# Autodesk Inventor assembly: Tamale - V1
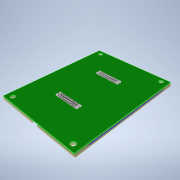
[picture p0: Inventor's stored thumbnail of the model, 180x180]
Saved by Autodesk Inventor 2022 (Build 260153000, 153)
## iProperties
Created: 2022-02-01
Part Number: Tamale - V1
Document SubType Name: Assembly
Designer: Caleb
Author: Caleb
## Documents named in this file (6)
- C:\Users\Caleb\Desktop\nebraska-silicon-lab\Hardware\ETL\modules\tamale\Tamale - V1p1.iam
- C:\Users\Caleb\Desktop\nebraska-silicon-lab\Hardware\ETL\modules\etl standard baseplate with cutouts.ipt
- C:\Users\Caleb\Desktop\nebraska-silicon-lab\Hardware\ETL\modules\tamale\BBM.iam
- C:\Users\Caleb\Desktop\nebraska-silicon-lab\Hardware\ETL\modules\tamale\Wirebond.ipt
- C:\Users\Caleb\Desktop\nebraska-silicon-lab\Hardware\ETL\modules\tamale\Mock Module PCB - V2p1.iam
- C:\Users\Caleb\Desktop\nebraska-silicon-lab\Hardware\ETL\modules\tamale\Short Wirebond.ipt
## Components (290 placed, 5 different names)
1. etl standard baseplate with cutouts:1 — Mate:7, Flush:5, Flush:6
2. BBM:1 [sub-assembly] — Mate:2, Angle:2, Flush:1, Flush:4, Mate:5, Mate:7, Mate:8
3. BBM:2 [sub-assembly] — Mate:3, Angle:1, Flush:2, Flush:4
4. BBM:3 [sub-assembly] — Mate:1, Angle:3, Flush:1, Flush:3, Mate:5, Mate:6
5. BBM:4 [sub-assembly] — Mate:4, Angle:4, Flush:2, Flush:3, Mate:6
6. Mock Module PCB - V2p1:1 [sub-assembly] — Mate:1, Mate:2, Mate:3, Mate:4, Angle:1, Angle:2, Angle:3, Angle:4, Flush:5, Flush:6
7. Wirebond:1 — Mate:8
8. Wirebond:2
9. Wirebond:3
10. Wirebond:4
11. Wirebond:5
12. Wirebond:6
13. Wirebond:7
14. Wirebond:8
15. Wirebond:9
16. Wirebond:10
17. Wirebond:11
18. Wirebond:12
19. Wirebond:13
20. Wirebond:14
21. Wirebond:15
22. Wirebond:16
23. Wirebond:17
24. Wirebond:18
25. Wirebond:19
26. Wirebond:20
27. Wirebond:21
28. Wirebond:22
29. Wirebond:23
30. Wirebond:24
31. Wirebond:25
32. Wirebond:26
33. Wirebond:27
34. Wirebond:28
35. Wirebond:29
36. Wirebond:30
37. Wirebond:31
38. Wirebond:32
39. Wirebond:33
40. Wirebond:34
41. Wirebond:35
42. Wirebond:36
43. Wirebond:37
44. Wirebond:38
45. Wirebond:39
46. Wirebond:40
47. Wirebond:41
48. Wirebond:42
49. Wirebond:43
50. Wirebond:44
51. Wirebond:45
52. Wirebond:46
53. Wirebond:47
54. Wirebond:48
55. Wirebond:49
56. Wirebond:50
57. Wirebond:51
58. Wirebond:52
59. Wirebond:53
60. Wirebond:54
61. Wirebond:55
62. Wirebond:56
63. Wirebond:57
64. Wirebond:58
65. Wirebond:59
66. Wirebond:60
67. Wirebond:61
68. Wirebond:62
69. Wirebond:63
70. Wirebond:64
71. Wirebond:65
72. Wirebond:66
73. Wirebond:67
74. Wirebond:68
75. Wirebond:69
76. Wirebond:70
77. Wirebond:71
78. Wirebond:72
79. Wirebond:73
80. Wirebond:74
81. Wirebond:75
82. Wirebond:76
83. Wirebond:77
84. Wirebond:78
85. Wirebond:79
86. Wirebond:80
87. Wirebond:81
88. Wirebond:82
89. Wirebond:83
90. Wirebond:84
91. Wirebond:85
92. Wirebond:86
93. Wirebond:87
94. Wirebond:88
95. Wirebond:89
96. Wirebond:90
97. Wirebond:91
98. Wirebond:92
99. Wirebond:93
100. Wirebond:94
101. Wirebond:95
102. Wirebond:96
103. Wirebond:97
104. Wirebond:98
105. Wirebond:99
106. Wirebond:100
107. Wirebond:101
108. Wirebond:102
109. Wirebond:103
110. Wirebond:104
111. Wirebond:105
112. Wirebond:106
113. Wirebond:107
114. Wirebond:108
115. Wirebond:109
116. Wirebond:110
117. Wirebond:111
118. Wirebond:112
119. Wirebond:113
120. Wirebond:114
121. Wirebond:115
122. Wirebond:116
123. Wirebond:117
124. Wirebond:118
125. Wirebond:119
126. Wirebond:120
127. Wirebond:121
128. Wirebond:122
129. Wirebond:123
130. Wirebond:124
131. Wirebond:125
132. Wirebond:126
133. Wirebond:127
134. Wirebond:128
135. Wirebond:129
136. Wirebond:130
137. Wirebond:131
138. Wirebond:132
139. Wirebond:133
140. Wirebond:134
141. Wirebond:135
142. Wirebond:136
143. Wirebond:137
144. Wirebond:138
145. Wirebond:139
146. Wirebond:140
147. Wirebond:141
148. Wirebond:142
149. Wirebond:143
150. Wirebond:144
151. Wirebond:145
152. Wirebond:146
153. Wirebond:147
154. Wirebond:148
155. Wirebond:149
156. Wirebond:150
157. Wirebond:151
158. Wirebond:152
159. Wirebond:153
160. Wirebond:154
161. Wirebond:155
162. Wirebond:156
163. Wirebond:157
164. Wirebond:158
165. Wirebond:159
166. Wirebond:160
167. Wirebond:161
168. Wirebond:162
169. Wirebond:163
170. Wirebond:164
171. Wirebond:165
172. Wirebond:166
173. Wirebond:167
174. Wirebond:168
175. Wirebond:169
176. Wirebond:170
177. Wirebond:171
178. Wirebond:172
179. Wirebond:173
180. Wirebond:174
181. Wirebond:175
182. Wirebond:176
183. Wirebond:177
184. Wirebond:178
185. Wirebond:179
186. Wirebond:180
187. Wirebond:181
188. Wirebond:182
189. Wirebond:183
190. Wirebond:184
191. Wirebond:185
192. Wirebond:186
193. Wirebond:187
194. Wirebond:188
195. Wirebond:189
196. Wirebond:190
197. Wirebond:191
198. Wirebond:192
199. Wirebond:193
200. Wirebond:194
201. Wirebond:195
202. Wirebond:196
203. Wirebond:197
204. Wirebond:198
205. Wirebond:199
206. Wirebond:200
207. Wirebond:201
208. Wirebond:202
209. Wirebond:203
210. Wirebond:204
211. Wirebond:205
212. Wirebond:206
213. Wirebond:207
214. Wirebond:208
215. Wirebond:209
216. Wirebond:210
217. Wirebond:211
218. Wirebond:212
219. Wirebond:213
220. Short Wirebond:1
221. Short Wirebond:2
222. Short Wirebond:3
223. Short Wirebond:4
224. Short Wirebond:5
225. Short Wirebond:6
226. Short Wirebond:7
227. Short Wirebond:8
228. Short Wirebond:9
229. Short Wirebond:10
230. Short Wirebond:11
231. Short Wirebond:12
232. Short Wirebond:13
233. Short Wirebond:14
234. Short Wirebond:15
235. Short Wirebond:16
236. Short Wirebond:17
237. Short Wirebond:18
238. Short Wirebond:19
239. Short Wirebond:20
240. Short Wirebond:21
241. Short Wirebond:22
242. Short Wirebond:23
243. Short Wirebond:24
244. Short Wirebond:25
245. Short Wirebond:26
246. Short Wirebond:27
247. Short Wirebond:28
248. Short Wirebond:29
249. Short Wirebond:30
250. Short Wirebond:31
251. Short Wirebond:32
252. Short Wirebond:33
253. Short Wirebond:34
254. Short Wirebond:35
255. Short Wirebond:36
256. Short Wirebond:37
257. Short Wirebond:38
258. Short Wirebond:39
259. Short Wirebond:40
260. Short Wirebond:41
261. Short Wirebond:42
262. Short Wirebond:43
263. Short Wirebond:44
264. Short Wirebond:45
265. Short Wirebond:46
266. Short Wirebond:47
267. Short Wirebond:48
268. Short Wirebond:49
269. Short Wirebond:50
270. Short Wirebond:51
271. Short Wirebond:52
272. Short Wirebond:53
273. Short Wirebond:54
274. Short Wirebond:55
275. Short Wirebond:56
276. Short Wirebond:57
277. Short Wirebond:58
278. Short Wirebond:59
279. Short Wirebond:60
280. Short Wirebond:61
281. Short Wirebond:62
282. Short Wirebond:63
283. Short Wirebond:64
284. Short Wirebond:65
285. Short Wirebond:66
286. Short Wirebond:67
287. Short Wirebond:68
288. Short Wirebond:69
289. Short Wirebond:70
290. Short Wirebond:71
## Component patterns: (142 elements, first: Wirebond:1), (71 elements, first: Wirebond:143), (71 elements, first: Short Wirebond:1)
## Relationships (18: Mate 8, Flush 6, Angle 4)
- Mate:1: BBM:3 ↔ Mock Module PCB - V2p1:1
- Mate:2: BBM:1 ↔ Mock Module PCB - V2p1:1
- Mate:3: BBM:2 ↔ Mock Module PCB - V2p1:1
- Mate:4: BBM:4 ↔ Mock Module PCB - V2p1:1
- Angle:1 (0 deg): BBM:2 ↔ Mock Module PCB - V2p1:1
- Angle:2 (0 deg): BBM:1 ↔ Mock Module PCB - V2p1:1
- Angle:3 (0 deg): BBM:3 ↔ Mock Module PCB - V2p1:1
- Angle:4 (0 deg): BBM:4 ↔ Mock Module PCB - V2p1:1
- Flush:1: BBM:1 ↔ BBM:3
- Flush:2: BBM:2 ↔ BBM:4
- Flush:3: BBM:3 ↔ BBM:4
- Flush:4: BBM:1 ↔ BBM:2
- Mate:5 (0.2 mm): BBM:1 ↔ BBM:3
- Mate:6 (0.2 mm): BBM:3 ↔ BBM:4
- Mate:7: etl standard baseplate with cutouts:1 ↔ BBM:1
- Flush:5: etl standard baseplate with cutouts:1 ↔ Mock Module PCB - V2p1:1
- Flush:6 (-0.25 mm): etl standard baseplate with cutouts:1 ↔ Mock Module PCB - V2p1:1
- Mate:8: BBM:1 ↔ Wirebond:1
